# Autodesk Inventor assembly: door2_cover
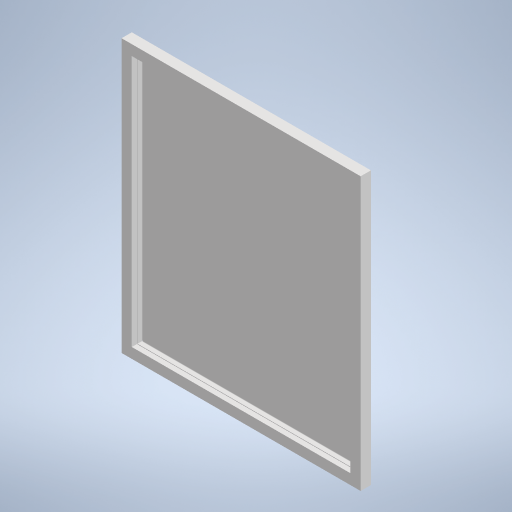
[picture p0: Inventor's stored thumbnail of the model, 512x512]
Saved by Autodesk Inventor 2023.5 (Build 275446000, 446)
## iProperties
Created: 2025-04-17
Part Number: door2_cover
Document SubType Name: Assembly
Designer: LENOVO
Author: LENOVO
## Documents named in this file (4)
- E:\filedata\invertorfile\tudien\door2_cover.iam
- E:\filedata\invertorfile\tudien\door2.ipt
- E:\filedata\invertorfile\tudien\coverdoor2.ipt
- E:\filedata\invertorfile\tudien\Handle 160 mm\Handle 160 mm.ipt
## Components (3 placed, 3 different names)
1. door2:1 — Mate:1, Mate:2, Flush:1, Mate:3, Flush:2, Flush:3
2. coverdoor2:1 — Mate:1, Mate:2, Flush:1
3. Handle 160 mm:1 — Mate:3, Flush:2, Flush:3
## Relationships (6: Mate 3, Flush 3)
- Mate:1: door2:1 ↔ coverdoor2:1
- Mate:2: door2:1 ↔ coverdoor2:1
- Flush:1: door2:1 ↔ coverdoor2:1
- Mate:3: door2:1 ↔ Handle 160 mm:1
- Flush:2: door2:1 ↔ Handle 160 mm:1
- Flush:3 (211 mm): door2:1 ↔ Handle 160 mm:1
